# Autodesk Inventor assembly: Assembly1
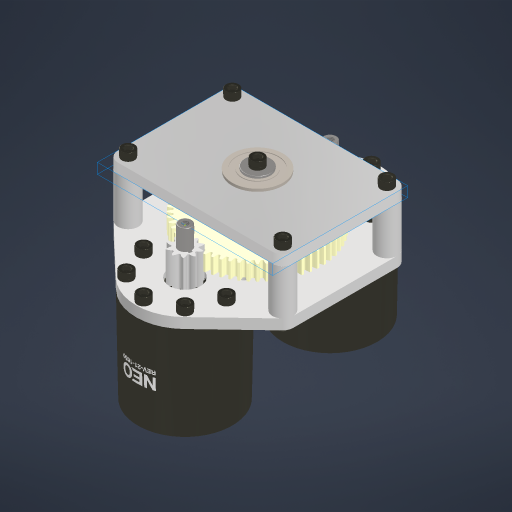
[picture p0: Inventor's stored thumbnail of the model, 512x512]
Saved by Autodesk Inventor 2024.3 (Build 283343000, 343)
## iProperties
Created: 2024-07-14
Part Number: Assembly1
Document SubType Name: Assembly
Designer: kaito
Author: kaito
## Documents named in this file (13)
- C:\Users\kaito\OneDrive\Documents\GitHub\1622-2024-Assignments\Kaito Kubota-Valme\Gearbox 2\Assembly1.iam
- C:\Users\kaito\OneDrive\Documents\GitHub\1622-2024-Assignments\Kaito Kubota-Valme\Gearbox 2\Bottom Plate.ipt
- C:\Users\kaito\OneDrive\Documents\GitHub\1622-2024-Assignments\Kaito Kubota-Valme\Gearbox 2\Top Plate.ipt
- C:\Users\kaito\OneDrive\Documents\GitHub\1622-2024-Assignments\Kaito Kubota-Valme\Gearbox 2\REV-21-1650-V1.1.ipt
- C:\Users\kaito\OneDrive\Desktop\Gearbox 2\REV-21-1998\REV-21-1998\REV-21-1998.ipt
- C:\Users\kaito\OneDrive\Documents\Inventor\Gearbox 1\Hex Bearing\Hex Bearing\Hex Bearing.ipt
- C:\Users\kaito\Downloads\WCP-0720 (1)\WCP-0720 (1)\WCP-0720 (1).ipt
- C:\Users\kaito\Downloads\WCP-0973 (1)\WCP-0973 (1)\WCP-0973 (1).ipt
- C:\Users\kaito\OneDrive\Documents\GitHub\1622-2024-Assignments\Kaito Kubota-Valme\Gearbox 2\sTANDOFF.ipt
- C:\Users\kaito\Downloads\hex.ipt
- C:\Users\kaito\OneDrive\Desktop\COTS Library\Fasteners\Bolts\Socket-Head\10-32\COTS91251A340_Black-Oxide Alloy Steel Socket Head Screw.ipt
- C:\Users\kaito\OneDrive\Desktop\COTS Library\Fasteners\Washers\COTS_90107A029_316 Stainless Steel Washer.ipt
- C:\Users\kaito\OneDrive\Desktop\COTS Library\Fasteners\Bolts\Socket-Head\10-32\COTS_91251A352_1.5in Long_Black-Oxide Alloy Steel Socket Head.ipt
## Components (32 placed, 12 different names)
1. Bottom Plate:1 — Mate:1, Mate:2, Mate:3, Mate:4, Mate:5, Mate:6, Mate:7, Mate:8, Mate:9, Mate:10, Mate:11, Mate:12, Mate:28, Mate:29, Mate:32, Mate:34, Mate:37, Mate:38, Mate:42, Mate:43, Mate:44, Mate:45, Mate:46, Mate:47, Mate:48, Mate:49, Mate:50, Mate:51, Mate:52, Mate:53, Mate:54, Mate:55, Mate:56, Mate:57, Mate:58, Mate:59, Mate:60, Mate:61
2. Top Plate:1 — Mate:1, Mate:2, Mate:19, Mate:20, Mate:30, Mate:31, Mate:33, Mate:36, Mate:66, Mate:67, Mate:68, Mate:69, Mate:70, Mate:71, Mate:72, Mate:73
3. REV-21-1650-V1.1:1 — Mate:8, Mate:9, Mate:10, Mate:11, Mate:12, Mate:13, Mate:23
4. REV-21-1650-V1.1:2 — Mate:3, Mate:4, Mate:5, Mate:6, Mate:7, Mate:14, Mate:24
5. REV-21-1998:1 — Mate:14, Mate:24
6. REV-21-1998:2 — Mate:13, Mate:23
7. Hex Bearing:2 — Mate:19, Mate:20, Mate:27, Mate:41, Flush:2, Mate:63
8. WCP-0720 (1):1 — Mate:25, Mate:26, Flush:1, Mate:39, Mate:40
9. WCP-0973 (1):1 — Mate:25, Mate:26, Flush:1, Mate:27
10. sTANDOFF:2 — Mate:32, Mate:33
11. sTANDOFF:3 — Mate:29, Mate:30
12. sTANDOFF:4 — Mate:34, Mate:36
13. sTANDOFF:5 — Mate:28, Mate:31
14. Hex Bearing:3 — Mate:37, Mate:38, Mate:39, Mate:40
15. hex:1 — Mate:41, Flush:2, Mate:62, Mate:64
16. COTS91251A340_Black-Oxide Alloy Steel Socket Head Screw:1 — Mate:49, Mate:55
17. COTS91251A340_Black-Oxide Alloy Steel Socket Head Screw:2 — Mate:42
18. COTS91251A340_Black-Oxide Alloy Steel Socket Head Screw:3 — Mate:46, Mate:59
19. COTS91251A340_Black-Oxide Alloy Steel Socket Head Screw:4 — Mate:47, Mate:60
20. COTS91251A340_Black-Oxide Alloy Steel Socket Head Screw:5 — Mate:51, Mate:56
21. COTS91251A340_Black-Oxide Alloy Steel Socket Head Screw:6 — Mate:53, Mate:58
22. COTS91251A340_Black-Oxide Alloy Steel Socket Head Screw:7 — Mate:48, Mate:61
23. COTS91251A340_Black-Oxide Alloy Steel Socket Head Screw:8 — Mate:50, Mate:54
24. COTS91251A340_Black-Oxide Alloy Steel Socket Head Screw:9 — Mate:52, Mate:57
25. COTS91251A340_Black-Oxide Alloy Steel Socket Head Screw:11 — Mate:64, Mate:65
26. COTS91251A340_Black-Oxide Alloy Steel Socket Head Screw:12 — Mate:43, Mate:44
27. COTS91251A340_Black-Oxide Alloy Steel Socket Head Screw:13 — Mate:45
28. COTS_90107A029_316 Stainless Steel Washer:1 — Mate:62, Mate:63, Mate:65
29. COTS_91251A352_1.5in Long_Black-Oxide Alloy Steel Socket Head:1 — Mate:66, Mate:67
30. COTS_91251A352_1.5in Long_Black-Oxide Alloy Steel Socket Head:2 — Mate:70, Mate:73
31. COTS_91251A352_1.5in Long_Black-Oxide Alloy Steel Socket Head:3 — Mate:69, Mate:72
32. COTS_91251A352_1.5in Long_Black-Oxide Alloy Steel Socket Head:4 — Mate:68, Mate:71
## Relationships (68: Mate 66, Flush 2)
- Mate:1: Bottom Plate:1 ↔ Top Plate:1
- Mate:2: Bottom Plate:1 ↔ Top Plate:1
- Mate:3: Bottom Plate:1 ↔ REV-21-1650-V1.1:2
- Mate:4: Bottom Plate:1 ↔ REV-21-1650-V1.1:2
- Mate:5: Bottom Plate:1 ↔ REV-21-1650-V1.1:2
- Mate:6: Bottom Plate:1 ↔ REV-21-1650-V1.1:2
- Mate:7: Bottom Plate:1 ↔ REV-21-1650-V1.1:2
- Mate:8: Bottom Plate:1 ↔ REV-21-1650-V1.1:1
- Mate:9: Bottom Plate:1 ↔ REV-21-1650-V1.1:1
- Mate:10: Bottom Plate:1 ↔ REV-21-1650-V1.1:1
- Mate:11: Bottom Plate:1 ↔ REV-21-1650-V1.1:1
- Mate:12: Bottom Plate:1 ↔ REV-21-1650-V1.1:1
- Mate:13: REV-21-1650-V1.1:1 ↔ REV-21-1998:2
- Mate:14: REV-21-1650-V1.1:2 ↔ REV-21-1998:1
- Mate:19: Top Plate:1 ↔ Hex Bearing:2
- Mate:20: Top Plate:1 ↔ Hex Bearing:2
- Mate:23: REV-21-1650-V1.1:1 ↔ REV-21-1998:2
- Mate:24: REV-21-1650-V1.1:2 ↔ REV-21-1998:1
- Mate:25: WCP-0720 (1):1 ↔ WCP-0973 (1):1
- Mate:26: WCP-0720 (1):1 ↔ WCP-0973 (1):1
- Flush:1: WCP-0720 (1):1 ↔ WCP-0973 (1):1
- Mate:27: Hex Bearing:2 ↔ WCP-0973 (1):1
- Mate:28: Bottom Plate:1 ↔ sTANDOFF:5
- Mate:29: Bottom Plate:1 ↔ sTANDOFF:3
- Mate:30: Top Plate:1 ↔ sTANDOFF:3
- Mate:31: Top Plate:1 ↔ sTANDOFF:5
- Mate:32: Bottom Plate:1 ↔ sTANDOFF:2
- Mate:33: Top Plate:1 ↔ sTANDOFF:2
- Mate:34: Bottom Plate:1 ↔ sTANDOFF:4
- Mate:36: Top Plate:1 ↔ sTANDOFF:4
- Mate:37: Bottom Plate:1 ↔ Hex Bearing:3
- Mate:38: Bottom Plate:1 ↔ Hex Bearing:3
- Mate:39: WCP-0720 (1):1 ↔ Hex Bearing:3
- Mate:40: WCP-0720 (1):1 ↔ Hex Bearing:3
- Mate:41: Hex Bearing:2 ↔ hex:1
- Flush:2: Hex Bearing:2 ↔ hex:1
- Mate:42: Bottom Plate:1 ↔ COTS91251A340_Black-Oxide Alloy Steel Socket Head Screw:2
- Mate:43: Bottom Plate:1 ↔ COTS91251A340_Black-Oxide Alloy Steel Socket Head Screw:12
- Mate:44: Bottom Plate:1 ↔ COTS91251A340_Black-Oxide Alloy Steel Socket Head Screw:12
- Mate:45: Bottom Plate:1 ↔ COTS91251A340_Black-Oxide Alloy Steel Socket Head Screw:13
- Mate:46: Bottom Plate:1 ↔ COTS91251A340_Black-Oxide Alloy Steel Socket Head Screw:3
- Mate:47: Bottom Plate:1 ↔ COTS91251A340_Black-Oxide Alloy Steel Socket Head Screw:4
- Mate:48: Bottom Plate:1 ↔ COTS91251A340_Black-Oxide Alloy Steel Socket Head Screw:7
- Mate:49: Bottom Plate:1 ↔ COTS91251A340_Black-Oxide Alloy Steel Socket Head Screw:1
- Mate:50: Bottom Plate:1 ↔ COTS91251A340_Black-Oxide Alloy Steel Socket Head Screw:8
- Mate:51: Bottom Plate:1 ↔ COTS91251A340_Black-Oxide Alloy Steel Socket Head Screw:5
- Mate:52: Bottom Plate:1 ↔ COTS91251A340_Black-Oxide Alloy Steel Socket Head Screw:9
- Mate:53: Bottom Plate:1 ↔ COTS91251A340_Black-Oxide Alloy Steel Socket Head Screw:6
- Mate:54: Bottom Plate:1 ↔ COTS91251A340_Black-Oxide Alloy Steel Socket Head Screw:8
- Mate:55: Bottom Plate:1 ↔ COTS91251A340_Black-Oxide Alloy Steel Socket Head Screw:1
- Mate:56: Bottom Plate:1 ↔ COTS91251A340_Black-Oxide Alloy Steel Socket Head Screw:5
- Mate:57: Bottom Plate:1 ↔ COTS91251A340_Black-Oxide Alloy Steel Socket Head Screw:9
- Mate:58: Bottom Plate:1 ↔ COTS91251A340_Black-Oxide Alloy Steel Socket Head Screw:6
- Mate:59: Bottom Plate:1 ↔ COTS91251A340_Black-Oxide Alloy Steel Socket Head Screw:3
- Mate:60: Bottom Plate:1 ↔ COTS91251A340_Black-Oxide Alloy Steel Socket Head Screw:4
- Mate:61: Bottom Plate:1 ↔ COTS91251A340_Black-Oxide Alloy Steel Socket Head Screw:7
- Mate:62: hex:1 ↔ COTS_90107A029_316 Stainless Steel Washer:1
- Mate:63: Hex Bearing:2 ↔ COTS_90107A029_316 Stainless Steel Washer:1
- Mate:64: hex:1 ↔ COTS91251A340_Black-Oxide Alloy Steel Socket Head Screw:11
- Mate:65: COTS91251A340_Black-Oxide Alloy Steel Socket Head Screw:11 ↔ COTS_90107A029_316 Stainless Steel Washer:1
- Mate:66: Top Plate:1 ↔ COTS_91251A352_1.5in Long_Black-Oxide Alloy Steel Socket Head:1
- Mate:67: Top Plate:1 ↔ COTS_91251A352_1.5in Long_Black-Oxide Alloy Steel Socket Head:1
- Mate:68: Top Plate:1 ↔ COTS_91251A352_1.5in Long_Black-Oxide Alloy Steel Socket Head:4
- Mate:69: Top Plate:1 ↔ COTS_91251A352_1.5in Long_Black-Oxide Alloy Steel Socket Head:3
- Mate:70: Top Plate:1 ↔ COTS_91251A352_1.5in Long_Black-Oxide Alloy Steel Socket Head:2
- Mate:71: Top Plate:1 ↔ COTS_91251A352_1.5in Long_Black-Oxide Alloy Steel Socket Head:4
- Mate:72: Top Plate:1 ↔ COTS_91251A352_1.5in Long_Black-Oxide Alloy Steel Socket Head:3
- Mate:73: Top Plate:1 ↔ COTS_91251A352_1.5in Long_Black-Oxide Alloy Steel Socket Head:2
